# Autodesk Inventor assembly: Auto Chair
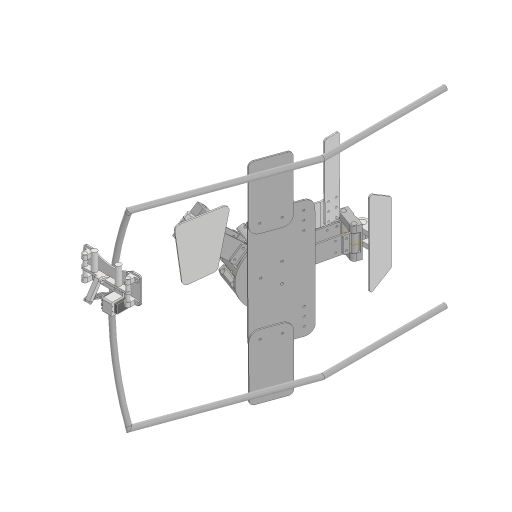
[picture p0: Inventor's stored thumbnail of the model, 512x512]
Saved by Autodesk Inventor 2024 (Build 280153000, 153)
## iProperties
Created: 2025-04-25
Part Number: Auto Chair
Document SubType Name: Assembly
Designer: Binara
Sending System: Autodesk Translation Framework v14.4.0.0
Preprocessor: ST-DEVELOPER v20.1
Title: Auto Chair.step
## Documents named in this file (28)
- Z:\Robotics\Inventor\Auto Chair\Auto Chair\Auto Chair.iam
- Z:\Robotics\Inventor\Auto Chair\Auto Chair\Chair Frame.ipt
- Z:\Robotics\Inventor\Auto Chair\Auto Chair\Leaf Spring.iam
- Z:\Robotics\Inventor\Auto Chair\Auto Chair\Arm Base.iam
- Z:\Robotics\Inventor\Auto Chair\Auto Chair\Part30.ipt
- Z:\Robotics\Inventor\Auto Chair\Auto Chair\Bolt.ipt
- Z:\Robotics\Inventor\Auto Chair\Auto Chair\Axle Joint.ipt
- Z:\Robotics\Inventor\Auto Chair\Auto Chair\Top Arm Plate.ipt
- Z:\Robotics\Inventor\Auto Chair\Auto Chair\Mg995 v1.ipt
- Z:\Robotics\Inventor\Auto Chair\Auto Chair\Servo Mount.ipt
- Z:\Robotics\Inventor\Auto Chair\Auto Chair\MG995_Gear2 v1.ipt
- Z:\Robotics\Inventor\Auto Chair\Auto Chair\Servo Small Arm.ipt
- Z:\Robotics\Inventor\Auto Chair\Auto Chair\Arm Link.ipt
- Z:\Robotics\Inventor\Auto Chair\Auto Chair\Servo Long Arm.ipt
- Z:\Robotics\Inventor\Auto Chair\Auto Chair\Endpoint.ipt
- Z:\Robotics\Inventor\Auto Chair\Auto Chair\Main Base.ipt
- Z:\Robotics\Inventor\Auto Chair\Auto Chair\Right Leaf.ipt
- Z:\Robotics\Inventor\Auto Chair\Auto Chair\Left Leaf.ipt
- Z:\Robotics\Inventor\Auto Chair\Upper Back Plate.ipt
- Z:\Robotics\Inventor\Auto Chair\Auto Chair\Servo Mount_MIR.ipt
- Z:\Robotics\Inventor\Auto Chair\Lower Back Plate.ipt
- Z:\Robotics\Inventor\Auto Chair\Large Pin.ipt
- Z:\Robotics\Inventor\Auto Chair\Neck Support\Neck Support.iam
- Z:\Robotics\Inventor\Auto Chair\LED Tower.ipt
- Z:\Robotics\Inventor\Auto Chair\LED disk.ipt
- Z:\Robotics\Inventor\Auto Chair\LED Diffuser.ipt
- Z:\Robotics\Inventor\Auto Chair\Angle.ipt
- Z:\Robotics\Inventor\Auto Chair\Lower Leaf.ipt
## Components (52 placed, 27 different names)
1. Chair Frame:1 — Tangent:1, Tangent:2
2. Leaf Spring:1 [sub-assembly]
3. Arm Base:1 [sub-assembly]
4. Part30 — Rotational:9, Rotational:10, Mate:11, Rotational:11, Rotational:12, Mate:16, Flush:9, Mate:17, Mate:20, Mate:21, Flush:10, Mate:22, Mate:23, Mate:24, Mate:25
5. Bolt:1 — Rotational:11, Flush:8, Mate:14
6. Axle Joint:1 — Mate:12, Flush:8, Mate:14
7. Axle Joint:2 — Mate:13, Mate:15
8. Bolt:2 — Rotational:12, Mate:15
9. Top Arm Plate:1 — Mate:13
10. Top Arm Plate:2 — Mate:12, Rigid:9
11. Axle Joint:3
12. Axle Joint:4
13. Mg995 v1:1 — Rigid:10, Rotational:13
14. Servo Mount:1 — Mate:16, Flush:9, Mate:17, Rigid:10
15. MG995_Gear2 v1:1 — Rotational:13, Rotational:14, Mate:18
16. Servo Small Arm:1 — Rotational:14, Mate:18, Rotational:15
17. Arm Link:1 — Rigid:9, Mate:19
18. Servo Long Arm:1 — Rotational:15, Mate:19
19. Bolt:5
20. Bolt:6
21. Endpoint:1 — Rotational:16, Angle:1
22. Bolt:3 — Rotational:9
23. Axle Joint:5
24. Axle Joint:6
25. Bolt:4 — Rotational:10
26. Top Arm Plate:3
27. Top Arm Plate:4
28. Axle Joint:7
29. Axle Joint:8
30. Mg995 v1:2
31. Servo Mount:2 — Mate:11
32. MG995_Gear2 v1:2
33. Servo Small Arm:2
34. Arm Link:2
35. Servo Long Arm:2
36. Bolt:7
37. Bolt:8
38. Endpoint:2 — Rotational:17, Angle:2
39. Main Base:1 — Rigid:12, Mate:20, Rigid:13, Mate:26, Mate:27, Mate:28
40. Right Leaf:1 — Tangent:1, Rigid:13
41. Left Leaf:1 — Rigid:12, Tangent:2
42. Upper Back Plate:1 — Rotational:16, Angle:1, Rotational:19
43. Servo Mount_MIR:1 — Mate:21, Flush:10, Mate:22
44. Lower Back Plate:1 — Rotational:17, Angle:2, Rotational:18
45. Large Pin:1 — Rotational:18
46. Large Pin:2 — Rotational:19
47. Neck Support:1 [sub-assembly]
48. LED Tower:1 — Mate:23, Mate:24, Mate:25, Rotational:20
49. LED disk:1 — Rotational:20, Rotational:21
50. LED Diffuser:1 — Rotational:21
51. Angle:1 — Mate:26, Mate:27, Mate:28, Rigid:14
52. Lower Leaf:1 — Rigid:14
## Relationships (76: Mate 28, RevoluteJoint 21, WeldJoint 13, Flush 10, Tangent 2, Angle 2)
- [RevoluteJoint]: Part30 ↔ Servo Mount:2
- [Flush] (15 mm): Axle Joint:3 ↔ Bolt:5
- [Mate]: Axle Joint:3 ↔ Bolt:5
- [Flush]: Axle Joint:3 ↔ Axle Joint:4
- [Mate]: Axle Joint:4 ↔ Bolt:6
- [Flush]: Bolt:5 ↔ Bolt:6
- [WeldJoint]: Top Arm Plate:1 ↔ Axle Joint:3
- [WeldJoint]: Top Arm Plate:2 ↔ Axle Joint:4
- [Mate]: Bolt:6 ↔ Endpoint:1
- [Mate]: Bolt:5 ↔ Endpoint:1
- [Flush]: Bolt:5 ↔ Endpoint:1
- [RevoluteJoint]: Axle Joint:1 ↔ Top Arm Plate:2
- [RevoluteJoint]: Axle Joint:2 ↔ Top Arm Plate:1
- [RevoluteJoint]: Bolt:7 ↔ Endpoint:2
- [RevoluteJoint]: Bolt:8 ↔ Endpoint:2
- [WeldJoint]: Top Arm Plate:3 ↔ Axle Joint:7
- [WeldJoint]: Top Arm Plate:4 ↔ Axle Joint:8
- [WeldJoint]: Axle Joint:6 ↔ Top Arm Plate:4
- [WeldJoint]: Axle Joint:5 ↔ Top Arm Plate:3
- [RevoluteJoint]: Arm Link:2 ↔ Servo Long Arm:2
- [WeldJoint]: Top Arm Plate:3 ↔ Arm Link:2
- [Mate]: Bolt:3 ↔ Axle Joint:5
- [Flush] (15.5 mm): Bolt:3 ↔ Axle Joint:5
- [WeldJoint]: Mg995 v1:2 ↔ Servo Mount:2
- [RevoluteJoint]: Mg995 v1:2 ↔ MG995_Gear2 v1:2
- [RevoluteJoint]: MG995_Gear2 v1:2 ↔ Servo Small Arm:2
- [Mate]: MG995_Gear2 v1:2 ↔ Servo Small Arm:2
- [Flush] (-15.01 mm): Axle Joint:7 ↔ Bolt:7
- [Mate]: Axle Joint:7 ↔ Bolt:7
- [Mate]: Axle Joint:8 ↔ Bolt:8
- [Flush] (15 mm): Axle Joint:8 ↔ Bolt:8
- [Mate]: Axle Joint:6 ↔ Bolt:4
- [Mate]: Servo Small Arm:2 ↔ Servo Long Arm:2
- Rotational:9 [RevoluteJoint]: Part30 ↔ Bolt:3
- Rotational:10 [RevoluteJoint]: Part30 ↔ Bolt:4
- Mate:11: Part30 ↔ Servo Mount:2
- Mate:12: Axle Joint:1 ↔ Top Arm Plate:2
- Mate:13: Axle Joint:2 ↔ Top Arm Plate:1
- Rotational:11 [RevoluteJoint]: Part30 ↔ Bolt:1
- Rotational:12 [RevoluteJoint]: Part30 ↔ Bolt:2
- Flush:8 (15.5 mm): Bolt:1 ↔ Axle Joint:1
- Mate:14: Bolt:1 ↔ Axle Joint:1
- Mate:15: Axle Joint:2 ↔ Bolt:2
- Rigid:9 [WeldJoint]: Top Arm Plate:2 ↔ Arm Link:1
- Mate:16: Part30 ↔ Servo Mount:1
- Flush:9: Part30 ↔ Servo Mount:1
- Mate:17: Part30 ↔ Servo Mount:1
- Rigid:10 [WeldJoint]: Mg995 v1:1 ↔ Servo Mount:1
- Rotational:13 [RevoluteJoint]: Mg995 v1:1 ↔ MG995_Gear2 v1:1
- Rotational:14 [RevoluteJoint]: MG995_Gear2 v1:1 ↔ Servo Small Arm:1
- Mate:18: MG995_Gear2 v1:1 ↔ Servo Small Arm:1
- Rotational:15 [RevoluteJoint]: Servo Small Arm:1 ↔ Servo Long Arm:1
- Mate:19: Arm Link:1 ↔ Servo Long Arm:1
- Rigid:12 [WeldJoint]: Main Base:1 ↔ Left Leaf:1
- Mate:20: Part30 ↔ Main Base:1
- Tangent:1: Chair Frame:1 ↔ Right Leaf:1
- Tangent:2: Chair Frame:1 ↔ Left Leaf:1
- Rigid:13 [WeldJoint]: Main Base:1 ↔ Right Leaf:1
- Rotational:16 [RevoluteJoint]: Endpoint:1 ↔ Upper Back Plate:1
- Angle:1 (0 deg): Endpoint:1 ↔ Upper Back Plate:1
- Mate:21: Part30 ↔ Servo Mount_MIR:1
- Flush:10: Part30 ↔ Servo Mount_MIR:1
- Mate:22: Part30 ↔ Servo Mount_MIR:1
- Rotational:17 [RevoluteJoint]: Endpoint:2 ↔ Lower Back Plate:1
- Angle:2 (20 deg): Endpoint:2 ↔ Lower Back Plate:1
- Rotational:18 [RevoluteJoint]: Lower Back Plate:1 ↔ Large Pin:1
- Rotational:19 [RevoluteJoint]: Upper Back Plate:1 ↔ Large Pin:2
- Mate:23: Part30 ↔ LED Tower:1
- Mate:24: Part30 ↔ LED Tower:1
- Mate:25: Part30 ↔ LED Tower:1
- Rotational:20 [RevoluteJoint]: LED Tower:1 ↔ LED disk:1
- Rotational:21 [RevoluteJoint]: LED disk:1 ↔ LED Diffuser:1
- Mate:26: Main Base:1 ↔ Angle:1
- Mate:27: Main Base:1 ↔ Angle:1
- Mate:28: Main Base:1 ↔ Angle:1
- Rigid:14 [WeldJoint]: Angle:1 ↔ Lower Leaf:1
## Named parameters: d2_d3 = 0 mm, d3_d4 = 0 deg, d9_d3 = 0 mm, d10_d4 = 0 mm, d20_d0 = 0 mm, d21_d1 = 21.902711 deg, d22_d2 = 0 mm, d23_d3 = -14.141842 deg, d24_d4 = 0 mm, d25_d5 = 0 mm, d26_d6 = 0 mm, d27_d7 = 0 mm, d28_d8 = 0 mm, d29_d9 = 92.251449 deg, d30_d10 = 0 mm, d31_d11 = 0 mm, d32_d12 = 15.5 mm, d33_d13 = 0 mm
